# Autodesk Inventor assembly: neo-7
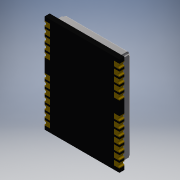
[picture p0: Inventor's stored thumbnail of the model, 180x180]
Saved by Autodesk Inventor 2016 (Build 200138000, 138)
## iProperties
Created: 2016-07-18
Part Number: neo-7
Document SubType Name: Assembly
Designer: Jonathan
Author: Jonathan
## Documents named in this file (3)
- C:\Users\Jonathan\Documents\Projects\anodePiShield\coincidenceCounter\cad\electronics\neo-7\neo-7.iam
- C:\Users\Jonathan\Documents\Projects\anodePiShield\coincidenceCounter\cad\electronics\neo-7\NEO-7.ipt
- C:\Users\Jonathan\Documents\Projects\anodePiShield\coincidenceCounter\cad\electronics\neo-7\cover.ipt
## Components (2 placed, 2 different names)
1. NEO-7:1 — Mate:1, Mate:2, Mate:3
2. cover:1 — Mate:1, Mate:2, Mate:3
## Relationships (3: Mate 3)
- Mate:1: NEO-7:1 ↔ cover:1
- Mate:2: NEO-7:1 ↔ cover:1
- Mate:3: NEO-7:1 ↔ cover:1
